# Autodesk Inventor assembly: sod_ii_complete
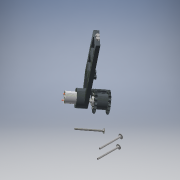
[picture p0: Inventor's stored thumbnail of the model, 180x180]
Saved by Autodesk Inventor 2016 (Build 200138000, 138)
## iProperties
Created: 2016-11-20
Part Number: sod_ii_complete
Document SubType Name: Assembly
Designer: hesaon
Author: hesaon
## Documents named in this file (18)
- D:\documents\SOD-II\cad\sod_ii_complete.iam
- D:\documents\SOD-II\cad\drive_sprocket_middle.ipt
- D:\documents\SOD-II\cad\outer_drive_sprocket.ipt
- D:\documents\SOD-II\cad\screw_Ka22x16.ipt
- D:\documents\SOD-II\cad\motor_axle_mounting_hub_6_mm.ipt
- D:\documents\SOD-II\cad\drive_sprocket_inner.ipt
- D:\documents\SOD-II\cad\screw12x3mm.ipt
- D:\documents\SOD-II\cad\washer3mm.ipt
- D:\documents\SOD-II\cad\tracks_center_ver2.ipt
- D:\documents\SOD-II\cad\tracks_outer.ipt
- D:\documents\SOD-II\cad\37D mm metal gearmotor.ipt
- D:\documents\SOD-II\cad\chassi_front_right.ipt
- D:\documents\SOD-II\cad\wagon_bolt.ipt
- D:\documents\SOD-II\cad\chassi_back_right.ipt
- D:\documents\SOD-II\cad\bolt90x6mm.ipt
- D:\documents\SOD-II\cad\washers\washer12mm.ipt
- D:\documents\SOD-II\cad\nuts\nut6mm.ipt
- D:\documents\SOD-II\cad\chassiconnector.ipt
## Components (73 placed, 17 different names)
1. drive_sprocket_middle:1 — Insert:1, Insert:2, Insert:16, Insert:17
2. outer_drive_sprocket:1 — Insert:1, Insert:2, Insert:3, Insert:4, Insert:5, Insert:6, Insert:7, Insert:8, Insert:9, Insert:10, Insert:11, Insert:12, Insert:13, Insert:14, Insert:43, Flush:1
3. screw_Ka22x16:1 — Insert:6
4. screw_Ka22x16:2 — Insert:4
5. screw_Ka22x16:3 — Insert:3
6. screw_Ka22x16:4 — Insert:7
7. screw_Ka22x16:5 — Insert:10
8. screw_Ka22x16:6 — Insert:9
9. screw_Ka22x16:7 — Insert:8
10. screw_Ka22x16:8 — Insert:5
11. screw_Ka22x16:9 — Insert:14
12. screw_Ka22x16:10 — Insert:11
13. screw_Ka22x16:11 — Insert:12
14. screw_Ka22x16:12 — Insert:13
15. motor_axle_mounting_hub_6_mm:1 — Insert:15, Mate:1, Insert:53
16. drive_sprocket_inner:1 — Insert:15, Mate:1, Insert:16, Insert:17, Insert:25, Insert:26, Insert:27, Insert:28, Insert:29, Insert:30, Insert:31, Insert:32, Insert:33, Insert:34, Insert:35, Insert:36, Insert:37, Insert:38, Insert:39, Insert:40, Insert:41, Insert:42, Insert:44, Insert:45
17. screw12x3mm:1 — Insert:20
18. screw12x3mm:2 — Insert:21
19. screw12x3mm:3 — Insert:22
20. screw12x3mm:4 — Insert:19
21. screw12x3mm:5 — Insert:23
22. screw12x3mm:6 — Insert:24
23. washer3mm:1 — Insert:20, Insert:25
24. washer3mm:2 — Insert:21, Insert:29
25. washer3mm:3 — Insert:22, Insert:28
26. washer3mm:4 — Insert:23, Insert:26
27. washer3mm:5 — Insert:19, Insert:27
28. washer3mm:6 — Insert:24, Insert:30
29. screw_Ka22x16:13 — Insert:40
30. screw_Ka22x16:14 — Insert:33
31. screw_Ka22x16:15 — Insert:34
32. screw_Ka22x16:16 — Insert:31
33. screw_Ka22x16:17 — Insert:39
34. screw_Ka22x16:18 — Insert:37
35. screw_Ka22x16:19 — Insert:42
36. screw_Ka22x16:20 — Insert:32
37. screw_Ka22x16:21 — Insert:36
38. screw_Ka22x16:22 — Insert:38
39. screw_Ka22x16:23 — Insert:41
40. screw_Ka22x16:24 — Insert:35
41. tracks_center_ver2:1 — Insert:45
42. tracks_center_ver2:2 — Insert:44
43. tracks_center_ver2:3 — Insert:43, Insert:48
44. tracks_outer:1 — Insert:48, Insert:50
45. tracks_outer:2 — Insert:49, Insert:50, Insert:51, Insert:52
46. tracks_outer:3 — Insert:49
47. screw_Ka22x16:25 — Insert:52
48. screw_Ka22x16:26 — Insert:51
49. 37D mm metal gearmotor:1 — Insert:53, Insert:54, Insert:55
50. chassi_front_right:1 — Insert:54, Insert:55, Insert:56, Insert:57, Insert:58, Insert:59, Insert:60, Insert:61, Mate:2, Flush:2, Flush:3, Insert:74, Insert:75
51. wagon_bolt:1
52. wagon_bolt:2 — Flush:1
53. wagon_bolt:3
54. screw12x3mm:7 — Insert:62
55. screw12x3mm:8 — Insert:64
56. screw12x3mm:9 — Insert:65
57. screw12x3mm:10 — Insert:67
58. screw12x3mm:11 — Insert:66
59. screw12x3mm:12 — Insert:63
60. washer3mm:7 — Insert:56, Insert:63
61. washer3mm:8 — Insert:57, Insert:64
62. washer3mm:9 — Insert:58, Insert:65
63. washer3mm:10 — Insert:61, Insert:67
64. washer3mm:11 — Insert:60, Insert:62
65. washer3mm:12 — Insert:59, Insert:66
66. chassi_back_right:1 — Mate:2, Flush:2, Flush:3, Insert:68, Insert:69, Angle:1, Angle:2
67. bolt90x6mm:1 — Insert:70, Insert:72
68. bolt90x6mm:2 — Insert:71, Insert:73
69. washer12mm:1 — Insert:68, Insert:70
70. washer12mm:2 — Insert:69, Insert:71
71. nut6mm:1 — Insert:72, Angle:2
72. nut6mm:2 — Insert:73, Angle:1
73. chassiconnector:1 — Insert:74, Insert:75
## Relationships (79: Insert 72, Flush 3, Mate 2, Angle 2)
- Insert:1: drive_sprocket_middle:1 ↔ outer_drive_sprocket:1
- Insert:2: drive_sprocket_middle:1 ↔ outer_drive_sprocket:1
- Insert:3: outer_drive_sprocket:1 ↔ screw_Ka22x16:3
- Insert:4: outer_drive_sprocket:1 ↔ screw_Ka22x16:2
- Insert:5: outer_drive_sprocket:1 ↔ screw_Ka22x16:8
- Insert:6: outer_drive_sprocket:1 ↔ screw_Ka22x16:1
- Insert:7: outer_drive_sprocket:1 ↔ screw_Ka22x16:4
- Insert:8: outer_drive_sprocket:1 ↔ screw_Ka22x16:7
- Insert:9: outer_drive_sprocket:1 ↔ screw_Ka22x16:6
- Insert:10: outer_drive_sprocket:1 ↔ screw_Ka22x16:5
- Insert:11: outer_drive_sprocket:1 ↔ screw_Ka22x16:10
- Insert:12: outer_drive_sprocket:1 ↔ screw_Ka22x16:11
- Insert:13: outer_drive_sprocket:1 ↔ screw_Ka22x16:12
- Insert:14: outer_drive_sprocket:1 ↔ screw_Ka22x16:9
- Insert:15: motor_axle_mounting_hub_6_mm:1 ↔ drive_sprocket_inner:1
- Mate:1: motor_axle_mounting_hub_6_mm:1 ↔ drive_sprocket_inner:1
- Insert:16: drive_sprocket_middle:1 ↔ drive_sprocket_inner:1
- Insert:17: drive_sprocket_middle:1 ↔ drive_sprocket_inner:1
- Insert:19: screw12x3mm:4 ↔ washer3mm:5
- Insert:20: screw12x3mm:1 ↔ washer3mm:1
- Insert:21: screw12x3mm:2 ↔ washer3mm:2
- Insert:22: screw12x3mm:3 ↔ washer3mm:3
- Insert:23: screw12x3mm:5 ↔ washer3mm:4
- Insert:24: screw12x3mm:6 ↔ washer3mm:6
- Insert:25: drive_sprocket_inner:1 ↔ washer3mm:1
- Insert:26: drive_sprocket_inner:1 ↔ washer3mm:4
- Insert:27: drive_sprocket_inner:1 ↔ washer3mm:5
- Insert:28: drive_sprocket_inner:1 ↔ washer3mm:3
- Insert:29: drive_sprocket_inner:1 ↔ washer3mm:2
- Insert:30: drive_sprocket_inner:1 ↔ washer3mm:6
- Insert:31: drive_sprocket_inner:1 ↔ screw_Ka22x16:16
- Insert:32: drive_sprocket_inner:1 ↔ screw_Ka22x16:20
- Insert:33: drive_sprocket_inner:1 ↔ screw_Ka22x16:14
- Insert:34: drive_sprocket_inner:1 ↔ screw_Ka22x16:15
- Insert:35: drive_sprocket_inner:1 ↔ screw_Ka22x16:24
- Insert:36: drive_sprocket_inner:1 ↔ screw_Ka22x16:21
- Insert:37: drive_sprocket_inner:1 ↔ screw_Ka22x16:18
- Insert:38: drive_sprocket_inner:1 ↔ screw_Ka22x16:22
- Insert:39: drive_sprocket_inner:1 ↔ screw_Ka22x16:17
- Insert:40: drive_sprocket_inner:1 ↔ screw_Ka22x16:13
- Insert:41: drive_sprocket_inner:1 ↔ screw_Ka22x16:23
- Insert:42: drive_sprocket_inner:1 ↔ screw_Ka22x16:19
- Insert:43 (-0.25 mm): outer_drive_sprocket:1 ↔ tracks_center_ver2:3
- Insert:44 (-0.25 mm): drive_sprocket_inner:1 ↔ tracks_center_ver2:2
- Insert:45 (-0.25 mm): drive_sprocket_inner:1 ↔ tracks_center_ver2:1
- Insert:48: tracks_center_ver2:3 ↔ tracks_outer:1
- Insert:49: tracks_outer:2 ↔ tracks_outer:3
- Insert:50: tracks_outer:1 ↔ tracks_outer:2
- Insert:51: tracks_outer:2 ↔ screw_Ka22x16:26
- Insert:52: tracks_outer:2 ↔ screw_Ka22x16:25
- Insert:53: motor_axle_mounting_hub_6_mm:1 ↔ 37D mm metal gearmotor:1
- Flush:1: outer_drive_sprocket:1 ↔ wagon_bolt:2
- Insert:54: 37D mm metal gearmotor:1 ↔ chassi_front_right:1
- Insert:55: 37D mm metal gearmotor:1 ↔ chassi_front_right:1
- Insert:56: chassi_front_right:1 ↔ washer3mm:7
- Insert:57: chassi_front_right:1 ↔ washer3mm:8
- Insert:58: chassi_front_right:1 ↔ washer3mm:9
- Insert:59: chassi_front_right:1 ↔ washer3mm:12
- Insert:60: chassi_front_right:1 ↔ washer3mm:11
- Insert:61: chassi_front_right:1 ↔ washer3mm:10
- Insert:62: screw12x3mm:7 ↔ washer3mm:11
- Insert:63: screw12x3mm:12 ↔ washer3mm:7
- Insert:64: screw12x3mm:8 ↔ washer3mm:8
- Insert:65: screw12x3mm:9 ↔ washer3mm:9
- Insert:66: screw12x3mm:11 ↔ washer3mm:12
- Insert:67: screw12x3mm:10 ↔ washer3mm:10
- Mate:2: chassi_front_right:1 ↔ chassi_back_right:1
- Flush:2: chassi_front_right:1 ↔ chassi_back_right:1
- Flush:3: chassi_front_right:1 ↔ chassi_back_right:1
- Insert:68: chassi_back_right:1 ↔ washer12mm:1
- Insert:69: chassi_back_right:1 ↔ washer12mm:2
- Insert:70: bolt90x6mm:1 ↔ washer12mm:1
- Insert:71: bolt90x6mm:2 ↔ washer12mm:2
- Insert:72 (1 mm): bolt90x6mm:1 ↔ nut6mm:1
- Insert:73 (1 mm): bolt90x6mm:2 ↔ nut6mm:2
- Angle:1 (0 deg): chassi_back_right:1 ↔ nut6mm:2
- Angle:2 (0 deg): chassi_back_right:1 ↔ nut6mm:1
- Insert:74: chassi_front_right:1 ↔ chassiconnector:1
- Insert:75: chassi_front_right:1 ↔ chassiconnector:1
